# Autodesk Inventor assembly: Assembly
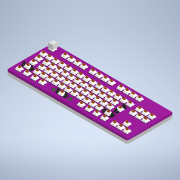
[picture p0: Inventor's stored thumbnail of the model, 180x180]
Saved by Autodesk Inventor 2022 (Build 260153000, 153)
## iProperties
Created: 2021-09-25
Part Number: Assembly
Document SubType Name: Weldment
Designer: shiok
Weld Material: Welded Aluminum-6061
Author: shiok
## Documents named in this file (5)
- C:\Users\Yazawa\Documents\GitHub\Keyboard_H\chassis\2022\Assembly.iam
- C:\Users\Yazawa\Documents\GitHub\Keyboard_H\chassis\2022\Base.ipt
- C:\Users\Yazawa\Documents\GitHub\Keyboard_H\chassis\2022\Plate.ipt
- C:\Users\Yazawa\Documents\GitHub\Keyboard_H\pcb\3D_model\step\keyboard_h.iam
- C:\Users\Yazawa\Documents\GitHub\Keyboard_H\chassis\2022\Cap.ipt
## Components (4 placed, 4 different names)
1. Plate:1 — メイト:2, 挿入:3, 挿入:4
2. keyboard_h:1 [sub-assembly] — メイト:1, 挿入:1, 挿入:2, メイト:2, 挿入:3, 挿入:4, メイト:3, メイト:4, メイト:5
3. Base:1 — メイト:1, 挿入:1, 挿入:2
4. Cap:1 — メイト:3, メイト:4, メイト:5
## Relationships (9: Mate 5, Insert 4)
- メイト:1 [Mate]: keyboard_h:1 ↔ Base:1
- 挿入:1 [Insert]: keyboard_h:1 ↔ Base:1
- 挿入:2 [Insert]: keyboard_h:1 ↔ Base:1
- メイト:2 [Mate]: Plate:1 ↔ keyboard_h:1
- 挿入:3 [Insert]: Plate:1 ↔ keyboard_h:1
- 挿入:4 [Insert]: Plate:1 ↔ keyboard_h:1
- メイト:3 [Mate]: keyboard_h:1 ↔ Cap:1
- メイト:4 [Mate]: keyboard_h:1 ↔ Cap:1
- メイト:5 [Mate]: keyboard_h:1 ↔ Cap:1
